# Autodesk Inventor assembly: ShakerAssembly
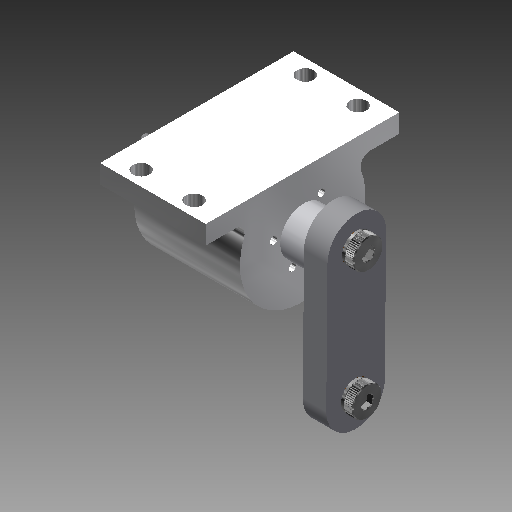
[picture p0: Inventor's stored thumbnail of the model, 512x512]
Saved by Autodesk Inventor 2017 (Build 210142000, 142)
## iProperties
Created: 2017-02-08
Part Number: ShakerAssembly
Document SubType Name: Assembly
Designer: Joseph
Author: Joseph
## Documents named in this file (8)
- D:\UMD Near Space\STAR\CAD\Mechanical\Subsystems\ShakerCAD\ShakerAssembly.iam
- C:\Users\qupec\Desktop\UMD Near Space\RockSat\ShakerCAD\MotorMount.ipt
- D:\UMD Near Space\STAR\CAD\Mechanical\Subsystems\ShakerCAD\Motor.ipt
- D:\UMD Near Space\STAR\CAD\Mechanical\Subsystems\ShakerCAD\MotorArm.ipt
- D:\UMD Near Space\STAR\CAD\Mechanical\Subsystems\ShakerCAD\RotationArm.ipt
- D:\UMD Near Space\STAR\CAD\Mechanical\Subsystems\ShakerCAD\Linkage.ipt
- D:\UMD Near Space\STAR\CAD\Mechanical\Subsystems\Motor Holder.ipt
- D:\UMD Near Space\STAR\CAD\Mechanical\Subsystems\ShakerCAD\Bearing correct.ipt
## Components (9 placed, 7 different names)
1. MotorMount:1 — Insert:1, Insert:2
2. Motor:1 — Insert:1, Insert:2, Rotational:1, Mate:2, Mate:3, Mate:4, Mate:5
3. MotorArm:1 — Rotational:1, Rotational:2
4. RotationArm:1 — Rotational:2, Mate:6, Mate:7
5. Linkage:1 — Mate:8, Mate:9, Flush:1, Flush:2
6. RotationArm:2 — Mate:10, Flush:3
7. Motor Holder:1 — Mate:2, Mate:3, Mate:4, Mate:5
8. Bearing correct:1 — Mate:6, Mate:7, Mate:8, Flush:2
9. Bearing correct:2 — Mate:9, Flush:1, Mate:10, Flush:3
## Relationships (16: Mate 9, Flush 3, Insert 2, RevoluteJoint 2)
- Insert:1: MotorMount:1 ↔ Motor:1
- Insert:2: MotorMount:1 ↔ Motor:1
- Rotational:1 [RevoluteJoint]: Motor:1 ↔ MotorArm:1
- Rotational:2 [RevoluteJoint]: MotorArm:1 ↔ RotationArm:1
- Mate:2: Motor:1 ↔ Motor Holder:1
- Mate:3: Motor:1 ↔ Motor Holder:1
- Mate:4: Motor:1 ↔ Motor Holder:1
- Mate:5: Motor:1 ↔ Motor Holder:1
- Mate:6: RotationArm:1 ↔ Bearing correct:1
- Mate:7: RotationArm:1 ↔ Bearing correct:1
- Mate:8: Linkage:1 ↔ Bearing correct:1
- Mate:9: Linkage:1 ↔ Bearing correct:2
- Flush:1: Linkage:1 ↔ Bearing correct:2
- Flush:2: Linkage:1 ↔ Bearing correct:1
- Mate:10: RotationArm:2 ↔ Bearing correct:2
- Flush:3: RotationArm:2 ↔ Bearing correct:2
